# Autodesk Inventor assembly: assembly
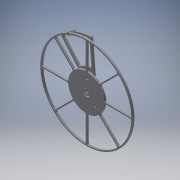
[picture p0: Inventor's stored thumbnail of the model, 180x180]
Saved by Autodesk Inventor 2019 (Build 230136000, 136)
## iProperties
Created: 2019-04-16
Part Number: assembly
Document SubType Name: Assembly
Designer: assman
Author: assman
## Documents named in this file (5)
- D:\Inventor\Projects\CatFeeder\Case\prototype\assembly.iam
- D:\Inventor\Projects\CatFeeder\Case\version6\motor_axis_join.ipt
- D:\Inventor\Projects\CatFeeder\Case\prototype\motor_apart.ipt
- D:\Inventor\Projects\CatFeeder\Case\prototype\floor.ipt
- D:\Inventor\Projects\CatFeeder\Case\prototype\upper.ipt
## Components (4 placed, 4 different names)
1. motor_apart:1 — Flush:1, Rotational:1
2. floor:1 — Flush:1
3. upper:1 — Rotational:1
4. motor_axis_join:1
## Relationships (2: Flush 1, RevoluteJoint 1)
- Flush:1: motor_apart:1 ↔ floor:1
- Rotational:1 [RevoluteJoint] (4 mm): motor_apart:1 ↔ upper:1
